# Autodesk Inventor assembly: Rocket Case
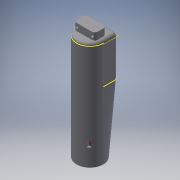
[picture p0: Inventor's stored thumbnail of the model, 180x180]
Saved by Autodesk Inventor 2019 (Build 230136000, 136)
## iProperties
Created: 2018-10-29
Part Number: Rocket Case
Document SubType Name: Assembly
Designer: Derek Fronek
Author: Derek Fronek
## Documents named in this file (4)
- C:\Users\Derek\OneDrive\Documents\Electrical Projects\Rocket team\Mechanical design\Rocket Case.iam
- C:\Users\Derek\OneDrive\Documents\Electrical Projects\Rocket team\Mechanical design\Rocket_Data_Logger v1.ipt
- C:\Users\Derek\OneDrive\Documents\Electrical Projects\Rocket team\Mechanical design\Bottom tube.ipt
- C:\Users\Derek\OneDrive\Documents\Electrical Projects\Rocket team\Mechanical design\Tube Top.ipt
## Components (3 placed, 3 different names)
1. Bottom tube:1 — Mate:1, Tangent:1, Tangent:2, Flush:1
2. Tube Top:1 — Flush:1
3. Rocket_Data_Logger v1:1 — Mate:1, Tangent:1, Tangent:2
## Relationships (4: Tangent 2, Mate 1, Flush 1)
- Mate:1: Bottom tube:1 ↔ Rocket_Data_Logger v1:1
- Tangent:1: Bottom tube:1 ↔ Rocket_Data_Logger v1:1
- Tangent:2: Bottom tube:1 ↔ Rocket_Data_Logger v1:1
- Flush:1: Bottom tube:1 ↔ Tube Top:1
